# Autodesk Inventor assembly: MGN15 Linear Rail 550mm - 4040 Assembly
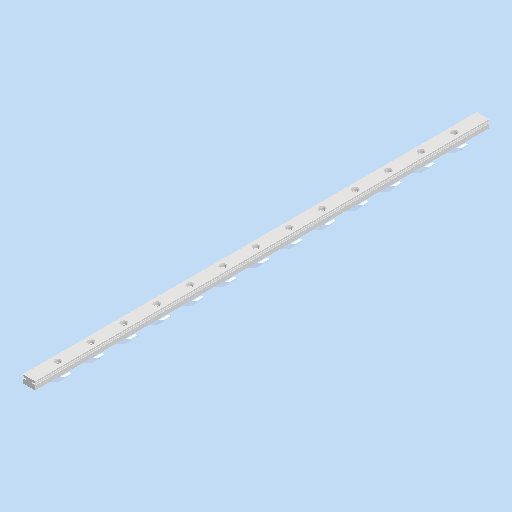
[picture p0: Inventor's stored thumbnail of the model, 512x512]
Saved by Autodesk Inventor 2023.2 (Build 272271000, 271)
## iProperties
Created: 2023-11-23
Part Number: MGN15 Linear Rail 550mm - 4040 Assembly
Document SubType Name: Assembly
Designer: Nils Bade
Author: Nils Bade
## Documents named in this file (4)
- C:\Users\nilsb\Documents\Inventor\Projektarbeit-Bade\RatRig_modified\MGN15 Linear Rail 550mm - 4040 Assembly.iam
- C:\Users\nilsb\Documents\Inventor\Projektarbeit-Bade\Schrauben\Cap Head Screw M3x12 v2.ipt
- C:\Users\nilsb\Documents\Inventor\Projektarbeit-Bade\RatRig_modified\MGN15 Linear Rail 550mm.ipt
- C:\Users\nilsb\Documents\Inventor\Projektarbeit-Bade\ITEM\item_Nutenstein 8 - M3_37359.ipt
## Components (27 placed, 3 different names)
1. MGN15 Linear Rail 550mm:1 — Passend:4, Passend:5, Passend:7
2. item_Nutenstein 8 - M3_37359:1 — Passend:3, Passend:6, Passend:7
3. Cap Head Screw M3x12 v2:1 — Passend:3, Passend:4, Passend:5
4. item_Nutenstein 8 - M3_37359:2
5. Cap Head Screw M3x12 v2:2
6. item_Nutenstein 8 - M3_37359:3
7. Cap Head Screw M3x12 v2:3
8. item_Nutenstein 8 - M3_37359:4
9. Cap Head Screw M3x12 v2:4
10. item_Nutenstein 8 - M3_37359:5
11. Cap Head Screw M3x12 v2:5
12. item_Nutenstein 8 - M3_37359:6
13. Cap Head Screw M3x12 v2:6
14. item_Nutenstein 8 - M3_37359:7
15. Cap Head Screw M3x12 v2:7
16. item_Nutenstein 8 - M3_37359:8
17. Cap Head Screw M3x12 v2:8
18. item_Nutenstein 8 - M3_37359:9
19. Cap Head Screw M3x12 v2:9
20. item_Nutenstein 8 - M3_37359:10
21. Cap Head Screw M3x12 v2:10
22. item_Nutenstein 8 - M3_37359:11
23. Cap Head Screw M3x12 v2:11
24. item_Nutenstein 8 - M3_37359:12
25. Cap Head Screw M3x12 v2:12
26. item_Nutenstein 8 - M3_37359:13
27. Cap Head Screw M3x12 v2:13
## Component patterns: (13 elements, first: item_Nutenstein 8 - M3_37359:1 + Cap Head Screw M3x12 v2:1)
## Relationships (5: Mate 5)
- Passend:3 [Mate]: item_Nutenstein 8 - M3_37359:1 ↔ Cap Head Screw M3x12 v2:1
- Passend:4 [Mate]: MGN15 Linear Rail 550mm:1 ↔ Cap Head Screw M3x12 v2:1
- Passend:5 [Mate]: MGN15 Linear Rail 550mm:1 ↔ Cap Head Screw M3x12 v2:1
- Passend:6 [Mate]: item_Nutenstein 8 - M3_37359:1
- Passend:7 [Mate] (4.5 mm): MGN15 Linear Rail 550mm:1 ↔ item_Nutenstein 8 - M3_37359:1
